# Autodesk Inventor assembly: Main
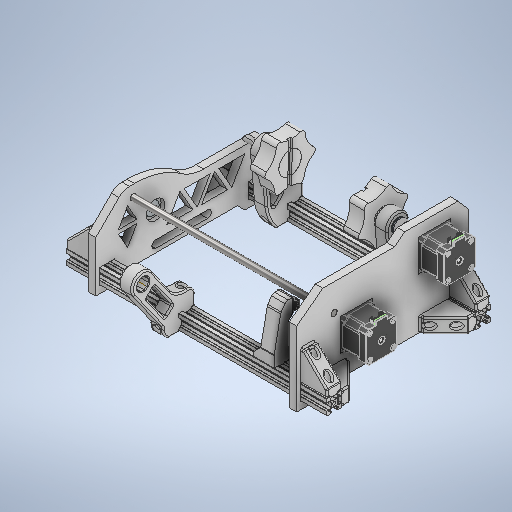
[picture p0: Inventor's stored thumbnail of the model, 512x512]
Saved by Autodesk Inventor 2025.3 (Build 293356030, 356C)
## iProperties
Created: 2025-09-01
Part Number: Main
Document SubType Name: Assembly
Designer: tvoko
Author: tvoko
## Documents named in this file (14)
- C:\Users\tvoko\Github\DIY-Coil-Winder\CAD\Main.iam
- C:\Users\tvoko\Github\DIY-Coil-Winder\CAD\2020-Profile.ipt
- C:\Users\tvoko\Github\DIY-Coil-Winder\CAD\Motor-Side.ipt
- C:\Users\tvoko\Github\DIY-Coil-Winder\CAD\Imports\NEMA 17 Stepper Motor 39mm-NEMA 17 Stepper Motor 39mm\barre T8 v1\barre T8 v1.ipt
- C:\Users\tvoko\Github\DIY-Coil-Winder\CAD\Imports\NEMA 17 Stepper Motor 39mm-NEMA 17 Stepper Motor 39mm\Creality Limit Switch\Creality Limit Switch.ipt
- C:\Users\tvoko\Github\DIY-Coil-Winder\CAD\Imports\NEMA 17 Stepper Motor 39mm-NEMA 17 Stepper Motor 39mm\F688ZZ Miniature Flanged Ball Bearing Low Detail\F688ZZ Miniature Flanged Ball Bearing Low Detail.ipt
- C:\Users\tvoko\Github\DIY-Coil-Winder\CAD\Imports\NEMA 17 Stepper Motor 39mm-NEMA 17 Stepper Motor 39mm\Flexible_Shaft_Coupling_5_to_8mm v7\Flexible_Shaft_Coupling_5_to_8mm v7.ipt
- C:\Users\tvoko\Github\DIY-Coil-Winder\CAD\Imports\NEMA 17 Stepper Motor 39mm-NEMA 17 Stepper Motor 39mm\NEMA 17 Stepper Motor 39mm-NEMA 17 Stepper Motor 39mm\NEMA 17 Stepper Motor 39mm-NEMA 17 Stepper Motor 39m.ipt
- C:\Users\tvoko\Github\DIY-Coil-Winder\CAD\Imports\M8x400-StainlessSteelRod.ipt
- C:\Users\tvoko\Github\DIY-Coil-Winder\CAD\Brace-Side.ipt
- C:\Users\tvoko\Github\DIY-Coil-Winder\CAD\Z-Endstop.ipt
- C:\Users\tvoko\Github\DIY-Coil-Winder\CAD\ToolLockAssy.iam
- C:\Users\tvoko\Github\DIY-Coil-Winder\CAD\Bearing-Holder.ipt
- C:\Users\tvoko\Github\DIY-Coil-Winder\CAD\Spool-Holder.ipt
## Components (22 placed, 13 different names)
1. 2020-Profile:1 — Mate:7, Mate:8, Mate:9, Mate:13, Mate:51
2. Motor-Side:1 — Mate:12, Mate:13, Mate:14, Mate:15, Mate:16, Mate:17, Mate:18, Mate:19, Mate:20, Flush:1, Flush:2, Flush:3, Flush:6, Flush:7, Flush:8, Flush:9, Flush:10, Flush:11, Flush:12
3. 2020-Profile:2 — Mate:10, Mate:11, Mate:12, Flush:1, Flush:4
4. barre T8 v1:1 — Mate:35, Mate:36, Mate:38
5. Creality Limit Switch:1 — Mate:40, Mate:41
6. F688ZZ Miniature Flanged Ball Bearing Low Detail:1 — Mate:38, Mate:39
7. Flexible_Shaft_Coupling_5_to_8mm v7:1 — Mate:2, Mate:3, Mate:35, Mate:36
8. NEMA 17 Stepper Motor 39mm-NEMA 17 Stepper Motor 39m:1 — Mate:2, Mate:3, Mate:14, Mate:15, Mate:16
9. NEMA 17 Stepper Motor 39mm-NEMA 17 Stepper Motor 39m:2 — Mate:17, Mate:18, Mate:19, Mate:42, Mate:43
10. Flexible_Shaft_Coupling_5_to_8mm v7:2 — Mate:42, Mate:43, Mate:44, Mate:45
11. F688ZZ Miniature Flanged Ball Bearing Low Detail:2 — Mate:46, Mate:49
12. M8x400-StainlessSteelRod:1 — Mate:20, Flush:8
13. Brace-Side:1 — Flush:2, Flush:3, Flush:4, Mate:39
14. Z-Endstop:1 — Flush:6, Flush:7, Mate:40, Mate:41
15. ToolLockAssy:1 [sub-assembly] — Mate:44, Mate:45, Mate:50, Mate:58
16. F688ZZ Miniature Flanged Ball Bearing Low Detail:5 — Mate:47, Mate:48, Mate:58
17. Bearing-Holder:1 — Mate:46, Mate:47, Mate:48, Mate:49, Mate:50, Mate:51
18. F688ZZ Miniature Flanged Ball Bearing Low Detail:6 — Mate:57
19. F688ZZ Miniature Flanged Ball Bearing Low Detail:7
20. Bearing-Holder:2 — Flush:9, Flush:10, Mate:56
21. Spool-Holder:1 — Flush:11, Flush:12
22. ToolLockAssy:2 [sub-assembly] — Mate:56, Mate:57
## Relationships (50: Mate 39, Flush 11)
- Mate:2: Flexible_Shaft_Coupling_5_to_8mm v7:1 ↔ NEMA 17 Stepper Motor 39mm-NEMA 17 Stepper Motor 39m:1
- Mate:3: Flexible_Shaft_Coupling_5_to_8mm v7:1 ↔ NEMA 17 Stepper Motor 39mm-NEMA 17 Stepper Motor 39m:1
- Mate:7: 2020-Profile:1
- Mate:8: 2020-Profile:1
- Mate:9: 2020-Profile:1
- Mate:10: 2020-Profile:2
- Mate:11: 2020-Profile:2
- Mate:12: Motor-Side:1 ↔ 2020-Profile:2
- Mate:13: 2020-Profile:1 ↔ Motor-Side:1
- Mate:14: Motor-Side:1 ↔ NEMA 17 Stepper Motor 39mm-NEMA 17 Stepper Motor 39m:1
- Mate:15: Motor-Side:1 ↔ NEMA 17 Stepper Motor 39mm-NEMA 17 Stepper Motor 39m:1
- Mate:16: Motor-Side:1 ↔ NEMA 17 Stepper Motor 39mm-NEMA 17 Stepper Motor 39m:1
- Mate:17: Motor-Side:1 ↔ NEMA 17 Stepper Motor 39mm-NEMA 17 Stepper Motor 39m:2
- Mate:18: Motor-Side:1 ↔ NEMA 17 Stepper Motor 39mm-NEMA 17 Stepper Motor 39m:2
- Mate:19: Motor-Side:1 ↔ NEMA 17 Stepper Motor 39mm-NEMA 17 Stepper Motor 39m:2
- Mate:20: Motor-Side:1 ↔ M8x400-StainlessSteelRod:1
- Mate:35: barre T8 v1:1 ↔ Flexible_Shaft_Coupling_5_to_8mm v7:1
- Mate:36: barre T8 v1:1 ↔ Flexible_Shaft_Coupling_5_to_8mm v7:1
- Flush:1: Motor-Side:1 ↔ 2020-Profile:2
- Flush:2: Motor-Side:1 ↔ Brace-Side:1
- Flush:3: Motor-Side:1 ↔ Brace-Side:1
- Mate:38: barre T8 v1:1 ↔ F688ZZ Miniature Flanged Ball Bearing Low Detail:1
- Flush:4: 2020-Profile:2 ↔ Brace-Side:1
- Mate:39: F688ZZ Miniature Flanged Ball Bearing Low Detail:1 ↔ Brace-Side:1
- Flush:6: Motor-Side:1 ↔ Z-Endstop:1
- Flush:7: Motor-Side:1 ↔ Z-Endstop:1
- Mate:40: Creality Limit Switch:1 ↔ Z-Endstop:1
- Mate:41: Creality Limit Switch:1 ↔ Z-Endstop:1
- Mate:42: NEMA 17 Stepper Motor 39mm-NEMA 17 Stepper Motor 39m:2 ↔ Flexible_Shaft_Coupling_5_to_8mm v7:2
- Mate:43: NEMA 17 Stepper Motor 39mm-NEMA 17 Stepper Motor 39m:2 ↔ Flexible_Shaft_Coupling_5_to_8mm v7:2
- Flush:8: Motor-Side:1 ↔ M8x400-StainlessSteelRod:1
- Mate:44: Flexible_Shaft_Coupling_5_to_8mm v7:2 ↔ ToolLockAssy:1
- Mate:45: Flexible_Shaft_Coupling_5_to_8mm v7:2 ↔ ToolLockAssy:1
- Mate:46: F688ZZ Miniature Flanged Ball Bearing Low Detail:2 ↔ Bearing-Holder:1
- Mate:47: F688ZZ Miniature Flanged Ball Bearing Low Detail:5 ↔ Bearing-Holder:1
- Mate:48: F688ZZ Miniature Flanged Ball Bearing Low Detail:5 ↔ Bearing-Holder:1
- Mate:49: F688ZZ Miniature Flanged Ball Bearing Low Detail:2 ↔ Bearing-Holder:1
- Mate:50: ToolLockAssy:1 ↔ Bearing-Holder:1
- Mate:51 (0.05 mm): 2020-Profile:1 ↔ Bearing-Holder:1
- [Mate]: F688ZZ Miniature Flanged Ball Bearing Low Detail:6 ↔ Bearing-Holder:2
- [Mate]: F688ZZ Miniature Flanged Ball Bearing Low Detail:7 ↔ Bearing-Holder:2
- [Mate]: F688ZZ Miniature Flanged Ball Bearing Low Detail:7 ↔ Bearing-Holder:2
- [Mate]: F688ZZ Miniature Flanged Ball Bearing Low Detail:6 ↔ Bearing-Holder:2
- Flush:9: Motor-Side:1 ↔ Bearing-Holder:2
- Flush:10: Motor-Side:1 ↔ Bearing-Holder:2
- Flush:11: Motor-Side:1 ↔ Spool-Holder:1
- Flush:12: Motor-Side:1 ↔ Spool-Holder:1
- Mate:56: Bearing-Holder:2 ↔ ToolLockAssy:2
- Mate:57: F688ZZ Miniature Flanged Ball Bearing Low Detail:6 ↔ ToolLockAssy:2
- Mate:58: ToolLockAssy:1 ↔ F688ZZ Miniature Flanged Ball Bearing Low Detail:5
## Named parameters: d65_d59 = 0 mm, d66_d60 = 0 mm, d67_d61 = 0 mm, d68_d62 = 0 mm
